# Autodesk Inventor assembly: ensamble montaje panel solar
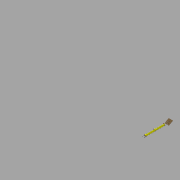
[picture p0: Inventor's stored thumbnail of the model, 180x180]
Saved by Autodesk Inventor 2014 (Build 180170000, 170)
## iProperties
Created: 2016-10-24
Part Number: ensamble montaje panel solar
Document SubType Name: Assembly
Designer: Cristian
Author: Cristian
## Documents named in this file (9)
- C:\Users\Cristian\Desktop\ANTENA MESH\ensamble montaje panel solar.iam
- C:\Users\Cristian\Desktop\ANTENA MESH\tubo base.ipt
- C:\Users\Cristian\Desktop\ANTENA MESH\ed30 panel solar.ipt
- C:\Users\Cristian\Desktop\ANTENA MESH\tubo corto.ipt
- C:\Users\Cristian\Desktop\ANTENA MESH\triangulo con anclajes.iam
- C:\Users\Cristian\Desktop\ANTENA MESH\anclaje panel 2 parte panel.ipt
- C:\Users\Cristian\Desktop\ANTENA MESH\anclaje panel 2 parte tubo.ipt
- C:\Users\Cristian\Desktop\ANTENA MESH\triangulo con anclajes sin aluc.iam
- C:\Users\Cristian\Desktop\ANTENA MESH\topes pata.ipt
## Components (17 placed, 8 different names)
1. tubo base:1 — Mate:1, Mate:4, Mate:33, Mate:47, Mate:78, Mate:81, Mate:92, Mate:94, Mate:95, Mate:96, Mate:98, Flush:23
2. tubo base:2 — Mate:2, Mate:3, Mate:34, Mate:40, Mate:50, Mate:79, Mate:80, Mate:91, Flush:21, Mate:99, Flush:24
3. tubo corto:1 — Mate:41, Mate:65, Mate:66
4. triangulo con anclajes:2 [sub-assembly] — Mate:33, Mate:34, Mate:46, Mate:47, Mate:90, Mate:93
5. tubo base:3 — Mate:40, Mate:41, Mate:46, Mate:49, Mate:97, Flush:22
6. triangulo con anclajes:4 [sub-assembly] — Mate:49, Mate:50, Mate:90
7. anclaje panel 2 parte tubo:1 — Mate:65, Mate:66, Mate:76, Mate:77
8. anclaje panel 2 parte panel:1 — Mate:76, Mate:77, Mate:87
9. anclaje panel 2 parte tubo:2 — Mate:79, Mate:80, Mate:82, Mate:84
10. anclaje panel 2 parte tubo:3 — Mate:78, Mate:81, Mate:85, Mate:86
11. anclaje panel 2 parte panel:2 — Mate:82, Mate:84, Mate:88, Flush:19, Flush:20
12. anclaje panel 2 parte panel:3 — Mate:85, Mate:86, Mate:89, Flush:19
13. ed30 panel solar:1 — Mate:87, Mate:88, Mate:89, Flush:20, Mate:96
14. triangulo con anclajes sin aluc:1 [sub-assembly] — Mate:91, Mate:92, Mate:93, Flush:21
15. topes pata:1 — Mate:98, Flush:23
16. topes pata:2 — Mate:99, Flush:24
17. topes pata:3 — Mate:97, Flush:22
## Relationships (43: Mate 37, Flush 6)
- Mate:1: tubo base:1
- Mate:2: tubo base:2
- Mate:3: tubo base:2
- Mate:4: tubo base:1
- Mate:33: tubo base:1 ↔ triangulo con anclajes:2
- Mate:34: tubo base:2 ↔ triangulo con anclajes:2
- Mate:40: tubo base:2 ↔ tubo base:3
- Mate:41: tubo corto:1 ↔ tubo base:3
- Mate:46: triangulo con anclajes:2 ↔ tubo base:3
- Mate:47: tubo base:1 ↔ triangulo con anclajes:2
- Mate:49: tubo base:3 ↔ triangulo con anclajes:4
- Mate:50: tubo base:2 ↔ triangulo con anclajes:4
- Mate:65: tubo corto:1 ↔ anclaje panel 2 parte tubo:1
- Mate:66: tubo corto:1 ↔ anclaje panel 2 parte tubo:1
- Mate:76: anclaje panel 2 parte tubo:1 ↔ anclaje panel 2 parte panel:1
- Mate:77: anclaje panel 2 parte tubo:1 ↔ anclaje panel 2 parte panel:1
- Mate:78: tubo base:1 ↔ anclaje panel 2 parte tubo:3
- Mate:79: tubo base:2 ↔ anclaje panel 2 parte tubo:2
- Mate:80: tubo base:2 ↔ anclaje panel 2 parte tubo:2
- Mate:81: tubo base:1 ↔ anclaje panel 2 parte tubo:3
- Mate:82: anclaje panel 2 parte tubo:2 ↔ anclaje panel 2 parte panel:2
- Mate:84: anclaje panel 2 parte tubo:2 ↔ anclaje panel 2 parte panel:2
- Mate:85: anclaje panel 2 parte tubo:3 ↔ anclaje panel 2 parte panel:3
- Mate:86: anclaje panel 2 parte tubo:3 ↔ anclaje panel 2 parte panel:3
- Mate:87: anclaje panel 2 parte panel:1 ↔ ed30 panel solar:1
- Mate:88: anclaje panel 2 parte panel:2 ↔ ed30 panel solar:1
- Mate:89: anclaje panel 2 parte panel:3 ↔ ed30 panel solar:1
- Flush:19: anclaje panel 2 parte panel:2 ↔ anclaje panel 2 parte panel:3
- Flush:20 (-70 mm): anclaje panel 2 parte panel:2 ↔ ed30 panel solar:1
- Mate:90 (1000 mm): triangulo con anclajes:2 ↔ triangulo con anclajes:4
- Mate:91: tubo base:2 ↔ triangulo con anclajes sin aluc:1
- Mate:92: tubo base:1 ↔ triangulo con anclajes sin aluc:1
- Mate:93: triangulo con anclajes:2 ↔ triangulo con anclajes sin aluc:1
- Flush:21 (200 mm): tubo base:2 ↔ triangulo con anclajes sin aluc:1
- Mate:94: tubo base:1
- Mate:95: tubo base:1
- Mate:96 (-120 mm): tubo base:1 ↔ ed30 panel solar:1
- Mate:97: tubo base:3 ↔ topes pata:3
- Mate:98: tubo base:1 ↔ topes pata:1
- Mate:99: tubo base:2 ↔ topes pata:2
- Flush:22 (-3 mm): tubo base:3 ↔ topes pata:3
- Flush:23 (-3 mm): tubo base:1 ↔ topes pata:1
- Flush:24 (-3 mm): tubo base:2 ↔ topes pata:2
